# Autodesk Inventor assembly: 0002_Truc_Z
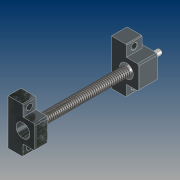
[picture p0: Inventor's stored thumbnail of the model, 180x180]
Saved by Autodesk Inventor 2021 (Build 250183000, 183)
## iProperties
Created: 2024-04-08
Part Number: 0002_Truc_Z
Document SubType Name: Assembly
Designer: Admin
Author: Admin
## Documents named in this file (6)
- C:\Users\Admin\Desktop\DO_AN_TOT_NGHIEP_2024\Mechanical\Design_in_3D\Version_2\0002_Truc_Z.iam
- C:\Users\Admin\Desktop\DO_AN_TOT_NGHIEP_2024\Mechanical\Design_in_3D\Library\Truc_vit_1405\Goi_do_A.ipt
- C:\Users\Admin\Desktop\DO_AN_TOT_NGHIEP_2024\Mechanical\Design_in_3D\Library\Truc_vit_1405\Goi_do_B.ipt
- C:\Users\Admin\Desktop\DO_AN_TOT_NGHIEP_2024\Mechanical\Design_in_3D\Library\Truc_vit_1405\Truc_vit.ipt
- C:\Users\Admin\Desktop\DO_AN_TOT_NGHIEP_2024\Mechanical\Design_in_3D\Library\Truc_vit_1405\Vong_chan.ipt
- C:\Users\Admin\Documents\Inventor\Content Center Files\R2021\en-US\BS EN ISO 4762\BS EN ISO 4762 - M3 x 6(1).ipt
## Components (8 placed, 5 different names)
1. Goi_do_A:1 — Insert:2, Flush:1
2. Goi_do_B:1 — Insert:1, Insert:3, Flush:1, Insert:4, Insert:5, Insert:6, Insert:7
3. Truc_vit:1 — Insert:1, Insert:2
4. Vong_chan:1 — Insert:3
5. BS EN ISO 4762 - Metric M3 x 6:1 — Insert:4
6. BS EN ISO 4762 - Metric M3 x 6:2 — Insert:5
7. BS EN ISO 4762 - Metric M3 x 6:3 — Insert:6
8. BS EN ISO 4762 - Metric M3 x 6:4 — Insert:7
## Relationships (8: Insert 7, Flush 1)
- Insert:1: Goi_do_B:1 ↔ Truc_vit:1
- Insert:2: Goi_do_A:1 ↔ Truc_vit:1
- Insert:3 (-1 mm): Goi_do_B:1 ↔ Vong_chan:1
- Flush:1: Goi_do_A:1 ↔ Goi_do_B:1
- Insert:4: Goi_do_B:1 ↔ BS EN ISO 4762 - Metric M3 x 6:1
- Insert:5: Goi_do_B:1 ↔ BS EN ISO 4762 - Metric M3 x 6:2
- Insert:6: Goi_do_B:1 ↔ BS EN ISO 4762 - Metric M3 x 6:3
- Insert:7: Goi_do_B:1 ↔ BS EN ISO 4762 - Metric M3 x 6:4
